# Autodesk Inventor assembly: segment2
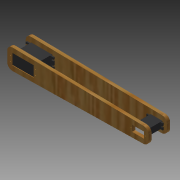
[picture p0: Inventor's stored thumbnail of the model, 180x180]
Saved by Autodesk Inventor 2013 (Build 170138000, 138)
## iProperties
Created: 2014-10-10
Part Number: segment2
Document SubType Name: Assembly
Designer: Masta
Author: Masta
## Documents named in this file (4)
- D:\DrOctopus\3D model\segment2.iam
- D:\DrOctopus\3D model\servo 13kg BMS-630MG.ipt
- D:\DrOctopus\3D model\segment2a.ipt
- D:\DrOctopus\3D model\serwo 2.8kg DS939HV.ipt
## Components (4 placed, 3 different names)
1. servo 13kg BMS-630MG:1 — Insert:4, Insert:5
2. segment2a:1 — Insert:3, Flush:1
3. segment2a:2 — Insert:3, Flush:1, Insert:4, Insert:5, Insert:6, Insert:7
4. serwo 2.8kg DS939HV:1 — Insert:6, Insert:7
## Relationships (6: Insert 5, Flush 1)
- Insert:3 (30 mm): segment2a:1 ↔ segment2a:2
- Flush:1: segment2a:1 ↔ segment2a:2
- Insert:4 (1 mm): servo 13kg BMS-630MG:1 ↔ segment2a:2
- Insert:5 (1 mm): servo 13kg BMS-630MG:1 ↔ segment2a:2
- Insert:6 (2 mm): segment2a:2 ↔ serwo 2.8kg DS939HV:1
- Insert:7 (2 mm): segment2a:2 ↔ serwo 2.8kg DS939HV:1
